# Autodesk Inventor assembly: LF_LapTimer-PCB
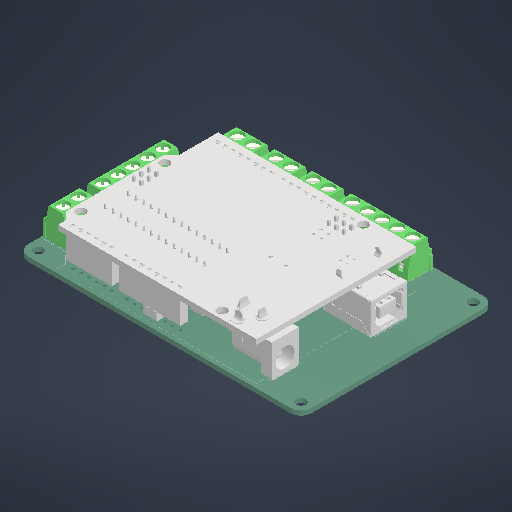
[picture p0: Inventor's stored thumbnail of the model, 512x512]
Saved by Autodesk Inventor 2026 (Build 300175000, 175)
## iProperties
Created: 2026-03-24
Part Number: LF_LapTimer-PCB
Document SubType Name: Assembly
Designer: vadim
Author: vadim
## Documents named in this file (7)
- C:\Users\vadim\GitHub\RoboCrew\RoboClash\LF-časomírá\_V2\FL-LapTimer\LF_LapTimer-PCB.iam
- C:\Users\vadim\GitHub\RoboCrew\RoboClash\LF-časomírá\_V2\Comp\LF_LAP_TIMER_PCB.ipt
- C:\Users\vadim\GitHub\RoboCrew\RoboClash\LF-časomírá\_V2\Comp\LF_LAP_TIMER_silkscreen.ipt
- C:\Users\vadim\GitHub\RoboCrew\RoboClash\LF-časomírá\_V2\Comp\180690550-9-1729128\1729128.iam
- C:\Users\vadim\GitHub\RoboCrew\RoboClash\LF-časomírá\_V2\Comp\180690877-9-1729131\1729131.iam
- C:\Users\vadim\GitHub\RoboCrew\RoboClash\LF-časomírá\_V2\Comp\2pin_header__02.ipt
- C:\Users\vadim\GitHub\RoboCrew\RoboClash\LF-časomírá\_V2\Comp\arduino uno.iam
## Components (12 placed, 6 different names)
1. LF_LAP_TIMER_PCB:1 — Tuhé:1, Tuhé:2, Tuhé:3, Tuhé:4, Tuhé:5, Tuhé:6, Tuhé:7, Tuhé:8, Tuhé:9, Tuhé:10
2. LF_LAP_TIMER_silkscreen:1 — Tuhé:1
3. 1729128:1 [sub-assembly] — Tuhé:2
4. 1729128:2 [sub-assembly] — Tuhé:3
5. 1729128:3 [sub-assembly] — Tuhé:4
6. 1729128:4 [sub-assembly] — Tuhé:8
7. 1729128:5 [sub-assembly] — Tuhé:7
8. 1729128:6 [sub-assembly] — Tuhé:5
9. 1729131:1 [sub-assembly] — Tuhé:6
10. 1729131:2 [sub-assembly] — Tuhé:9
11. 2pin_header__02:1 — Tuhé:10, Tuhé:11
12. arduino uno:1 [sub-assembly] — Tuhé:11
## Relationships (11: WeldJoint 11)
- Tuhé:1 [WeldJoint] (0.001 mm): LF_LAP_TIMER_PCB:1 ↔ LF_LAP_TIMER_silkscreen:1
- Tuhé:2 [WeldJoint] (-3.5 mm): LF_LAP_TIMER_PCB:1 ↔ 1729128:1
- Tuhé:3 [WeldJoint] (3.5 mm): LF_LAP_TIMER_PCB:1 ↔ 1729128:2
- Tuhé:4 [WeldJoint] (-3.5 mm): LF_LAP_TIMER_PCB:1 ↔ 1729128:3
- Tuhé:5 [WeldJoint] (3.5 mm): LF_LAP_TIMER_PCB:1 ↔ 1729128:6
- Tuhé:6 [WeldJoint] (3.5 mm): LF_LAP_TIMER_PCB:1 ↔ 1729131:1
- Tuhé:7 [WeldJoint] (3.5 mm): LF_LAP_TIMER_PCB:1 ↔ 1729128:5
- Tuhé:8 [WeldJoint] (3.5 mm): LF_LAP_TIMER_PCB:1 ↔ 1729128:4
- Tuhé:9 [WeldJoint] (3.5 mm): LF_LAP_TIMER_PCB:1 ↔ 1729131:2
- Tuhé:10 [WeldJoint] (3.25 mm): LF_LAP_TIMER_PCB:1 ↔ 2pin_header__02:1
- Tuhé:11 [WeldJoint] (-1 mm): 2pin_header__02:1 ↔ arduino uno:1
